# Autodesk Inventor assembly: head_link
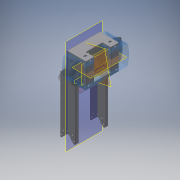
[picture p0: Inventor's stored thumbnail of the model, 180x180]
Saved by Autodesk Inventor 2018 (Build 220112000, 112)
## iProperties
Created: 2018-12-01
Part Number: head_link
Document SubType Name: Assembly
Designer: jaspe
Author: jaspe
## Documents named in this file (4)
- C:\Users\jaspe\bitbots_hardware\wolfgang\assembly\head\head_link.iam
- C:\Users\jaspe\bitbots_hardware\wolfgang\assembly\head\Logitech_C910_(interior).ipt
- C:\Users\jaspe\bitbots_hardware\wolfgang\assembly\head\camera_holder.ipt
- C:\Users\jaspe\bitbots_hardware\wolfgang\assembly\head\camera2.ipt
## Components (3 placed, 3 different names)
1. Logitech_C910_(interior):1 — Mate:1, Flush:1, Mate:8, Mate:9
2. camera_holder:1 — Mate:2, Mate:3, Flush:1, Mate:7, Mate:9, Flush:2, Flush:3
3. camera2:1 — Mate:1, Mate:2, Mate:3, Mate:4, Mate:5, Mate:7, Mate:8, Flush:4
## Relationships (13: Mate 9, Flush 4)
- Mate:1: Logitech_C910_(interior):1 ↔ camera2:1
- Mate:2: camera_holder:1 ↔ camera2:1
- Mate:3: camera_holder:1 ↔ camera2:1
- Flush:1: Logitech_C910_(interior):1 ↔ camera_holder:1
- Mate:4 (24 mm): camera2:1
- Mate:5: camera2:1
- Mate:7: camera_holder:1 ↔ camera2:1
- Mate:8: Logitech_C910_(interior):1 ↔ camera2:1
- Mate:9: Logitech_C910_(interior):1 ↔ camera_holder:1
- Flush:2 (16 mm): camera_holder:1
- Flush:3 (20 mm): camera_holder:1
- Flush:4 (-14.03 mm): camera2:1
- Mate:10
